# Autodesk Inventor assembly: Assy_CORE_board
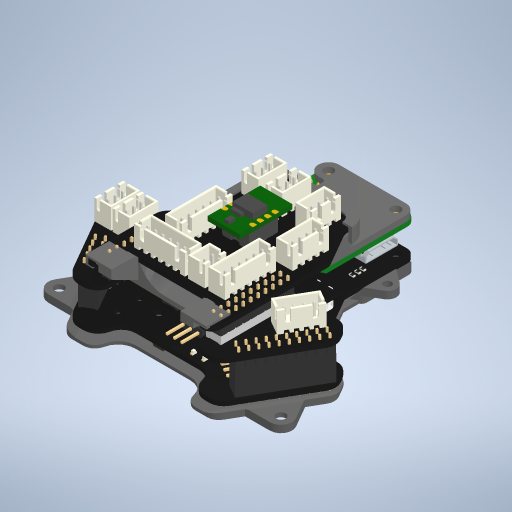
[picture p0: Inventor's stored thumbnail of the model, 512x512]
Saved by Autodesk Inventor 2024.1 (Build 281209000, 209)
## iProperties
Created: 2025-05-06
Part Number: Assy_CORE_board
Document SubType Name: Assembly
Designer: hibik
Author: hibik
## Documents named in this file (5)
- C:\Users\hibik\Documents\Robomech\RESCUE\ORCA\hard\flame_base\Assy_CORE_board.iam
- C:\Users\hibik\Documents\Robomech\RESCUE\ORCA\hard\board\CORE_model\CORE.iam
- C:\Users\hibik\Documents\Robomech\RESCUE\ORCA\hard\flame_base\CORE_board_setter.ipt
- C:\Users\hibik\Documents\Robomech\RESCUE\ORCA\hard\flame_base\CORE_board_middle_back.ipt
- C:\Users\hibik\Documents\Robomech\RESCUE\ORCA\hard\flame_base\CORE_board_middle_front.ipt
## Components (4 placed, 4 different names)
1. CORE_board_setter:1 — 挿入:1
2. CORE:1 [sub-assembly] — 挿入:1, 角度:1, 挿入:2, 角度:2, 挿入:3
3. CORE_board_middle_back:1 — 挿入:2, 角度:2
4. CORE_board_middle_front:1 — 挿入:3
## Relationships (5: Insert 3, Angle 2)
- 挿入:1 [Insert]: CORE_board_setter:1 ↔ CORE:1
- 角度:1 [Angle] (0 deg): CORE:1
- 挿入:2 [Insert]: CORE:1 ↔ CORE_board_middle_back:1
- 角度:2 [Angle] (0 deg): CORE:1 ↔ CORE_board_middle_back:1
- 挿入:3 [Insert]: CORE:1 ↔ CORE_board_middle_front:1
